# Autodesk Inventor assembly: uMule-UDaR
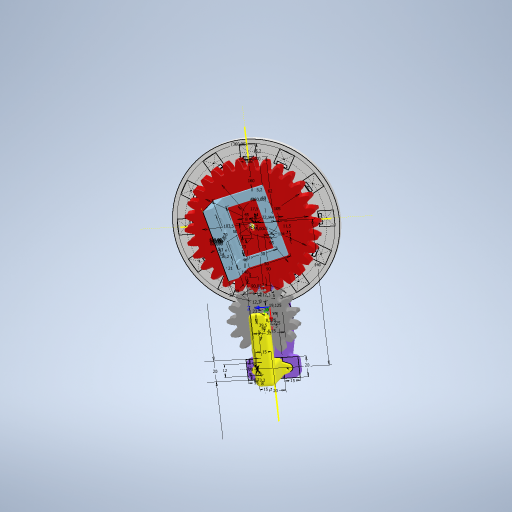
[picture p0: Inventor's stored thumbnail of the model, 512x512]
Saved by Autodesk Inventor 2024.2 (Build 282272000, 272)
## iProperties
Created: 2024-10-14
Part Number: uMule-UDaR
Document SubType Name: Assembly
Designer: owozn
Author: owozn
## Documents named in this file (9)
- C:\Users\owozn\Documents\Semestr 7\Inżynierka\Modele 3D\uMule-UDaR.iam
- C:\Users\owozn\Downloads\Part Studio 1 - Spur gear (15 teeth) (2)\Part Studio 1 - Spur gear (15 teeth) (2).ipt
- C:\Users\owozn\Documents\Semestr 7\Inżynierka\Modele 3D\Slip ring\SlipRing_with_Flange_22mm\SlipRing_with_Flange_22mm.ipt
- C:\Users\owozn\Documents\Semestr 7\Inżynierka\Modele 3D\uMule-UDaR-main_gear.ipt
- C:\Users\owozn\Documents\Semestr 7\Inżynierka\Modele 3D\uMule-UDaR-sensor.ipt
- C:\Users\owozn\Documents\Semestr 7\Inżynierka\Modele 3D\uMule_uchwyt-sens.ipt
- C:\Users\owozn\Documents\Semestr 7\Inżynierka\Modele 3D\tower-pro-mg90s-micro-servo-2.snapshot.3\Tower Pro MG90S Micro servo\Tower Pro MG90S Micro servo.ipt
- C:\Users\owozn\Documents\Semestr 7\Inżynierka\Modele 3D\uMule-uchwyt_servo.ipt
- C:\Users\owozn\Documents\Semestr 7\Inżynierka\Modele 3D\uMule-podstawka_czujnikiIR.ipt
## Components (8 placed, 8 different names)
1. Part Studio 1 - Spur gear (15 teeth) (2):1 — Zestawiające:1, Równoległe:1, Zestawiające:11, Zestawiające:12, Zestawiające:17
2. SlipRing_with_Flange_22mm:1 — Zestawiające:3, Zestawiające:7, Zestawiające:9, Zestawiające:14, Zestawiające:15
3. uMule-UDaR-main_gear:1 — Zestawiające:1, Zestawiające:3, Równoległe:1, Zestawiające:4, Zestawiające:5, Zestawiające:6, Zestawiające:15
4. uMule-UDaR-sensor:1 — Zestawiające:4, Zestawiające:5, Zestawiające:6
5. uMule_uchwyt-sens:1 — Zestawiające:7, Zestawiające:9, Zestawiające:13, Zestawiające:14, Równoległe:2, Zestawiające:18, Zestawiające:19, Zestawiające:20
6. Tower Pro MG90S Micro servo:1 — Zestawiające:11, Zestawiające:12, Zestawiające:13
7. uMule-uchwyt_servo:1 — Równoległe:2, Zestawiające:17, Zestawiające:18
8. uMule-podstawka_czujnikiIR:1 — Zestawiające:19, Zestawiające:20
## Relationships (18: Mate 16, Flush 2)
- Zestawiające:1 [Mate] (90 mm): Part Studio 1 - Spur gear (15 teeth) (2):1 ↔ uMule-UDaR-main_gear:1
- Zestawiające:3 [Mate] (2 mm): SlipRing_with_Flange_22mm:1 ↔ uMule-UDaR-main_gear:1
- Równoległe:1 [Flush]: Part Studio 1 - Spur gear (15 teeth) (2):1 ↔ uMule-UDaR-main_gear:1
- Zestawiające:4 [Mate]: uMule-UDaR-main_gear:1 ↔ uMule-UDaR-sensor:1
- Zestawiające:5 [Mate]: uMule-UDaR-main_gear:1 ↔ uMule-UDaR-sensor:1
- Zestawiające:6 [Mate]: uMule-UDaR-main_gear:1 ↔ uMule-UDaR-sensor:1
- Zestawiające:7 [Mate]: SlipRing_with_Flange_22mm:1 ↔ uMule_uchwyt-sens:1
- Zestawiające:9 [Mate]: SlipRing_with_Flange_22mm:1 ↔ uMule_uchwyt-sens:1
- Zestawiające:11 [Mate]: Part Studio 1 - Spur gear (15 teeth) (2):1 ↔ Tower Pro MG90S Micro servo:1
- Zestawiające:12 [Mate]: Part Studio 1 - Spur gear (15 teeth) (2):1 ↔ Tower Pro MG90S Micro servo:1
- Zestawiające:13 [Mate]: uMule_uchwyt-sens:1 ↔ Tower Pro MG90S Micro servo:1
- Zestawiające:14 [Mate]: SlipRing_with_Flange_22mm:1 ↔ uMule_uchwyt-sens:1
- Zestawiające:15 [Mate]: SlipRing_with_Flange_22mm:1 ↔ uMule-UDaR-main_gear:1
- Równoległe:2 [Flush]: uMule_uchwyt-sens:1 ↔ uMule-uchwyt_servo:1
- Zestawiające:17 [Mate]: Part Studio 1 - Spur gear (15 teeth) (2):1 ↔ uMule-uchwyt_servo:1
- Zestawiające:18 [Mate]: uMule_uchwyt-sens:1 ↔ uMule-uchwyt_servo:1
- Zestawiające:19 [Mate]: uMule_uchwyt-sens:1 ↔ uMule-podstawka_czujnikiIR:1
- Zestawiające:20 [Mate] (0.5 mm): uMule_uchwyt-sens:1 ↔ uMule-podstawka_czujnikiIR:1
## Named parameters: Finish1_Area = 68.2082
note: some values were not read from the file. Shown as the stored number, unit unknown: "Finish1_Area".
